# Autodesk Inventor assembly: Structure
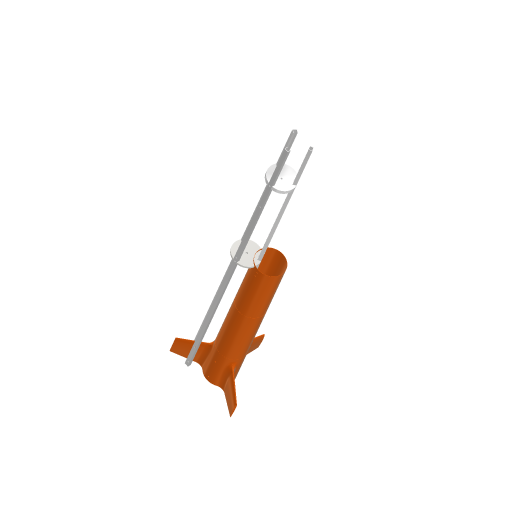
[picture p0: Inventor's stored thumbnail of the model, 512x512]
Saved by Autodesk Inventor 2024 (Build 280153000, 153)
## iProperties
Created: 2023-12-30
Part Number: Structure
Document SubType Name: Assembly
Designer: Jamie
Author: Jamie
## Documents named in this file (5)
- C:\Users\Jamie\Documents\Uni\DARE\Scrambler-2-CAD\Autodesk\Structure.iam
- C:\Users\Jamie\Documents\Uni\DARE\Scrambler-2-CAD\Autodesk\Engine bulkhead.ipt
- C:\Users\Jamie\Documents\Uni\DARE\Scrambler-2-CAD\Autodesk\Stringer.ipt
- C:\Users\Jamie\Documents\Uni\DARE\Scrambler-2-CAD\Autodesk\Parachute bulkhead.ipt
- C:\Users\Jamie\Documents\Uni\DARE\Scrambler-2-CAD\Autodesk\Engine skin glued.iam
## Components (6 placed, 4 different names)
1. Engine bulkhead:1 — Mate:16, Mate:17, Mate:18
2. Stringer:1 — Mate:12, Mate:16, Mate:23, Mate:26
3. Stringer:2 — Mate:13, Mate:15, Mate:17, Mate:24
4. Stringer:3 — Mate:11, Mate:18, Mate:25
5. Parachute bulkhead:1 — Mate:11, Mate:12, Mate:13, Mate:15, Mate:23, Mate:25
6. Engine skin glued:1 [sub-assembly] — Mate:24, Mate:26
## Relationships (11: Mate 11)
- Mate:11 (0.5 mm): Stringer:3 ↔ Parachute bulkhead:1
- Mate:12 (0.5 mm): Stringer:1 ↔ Parachute bulkhead:1
- Mate:13 (0.5 mm): Stringer:2 ↔ Parachute bulkhead:1
- Mate:15: Stringer:2 ↔ Parachute bulkhead:1
- Mate:16: Engine bulkhead:1 ↔ Stringer:1
- Mate:17: Engine bulkhead:1 ↔ Stringer:2
- Mate:18: Engine bulkhead:1 ↔ Stringer:3
- Mate:23: Stringer:1 ↔ Parachute bulkhead:1
- Mate:24: Stringer:2 ↔ Engine skin glued:1
- Mate:25: Stringer:3 ↔ Parachute bulkhead:1
- Mate:26: Stringer:1 ↔ Engine skin glued:1
